# Autodesk Inventor assembly: XL430-bracket
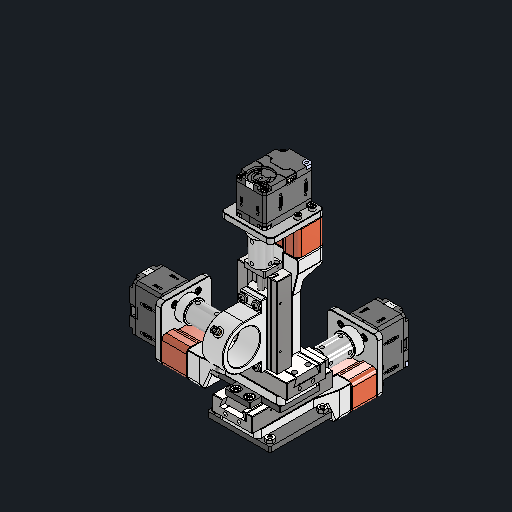
[picture p0: Inventor's stored thumbnail of the model, 512x512]
Saved by Autodesk Inventor 2027.1 (Build 311270010, 270A)
## iProperties
Created: 2025-05-28
Part Number: XL430-bracket
Document SubType Name: Assembly
Designer: kuzmin
Mass: 1365.19 g
Surface Area: 1309.73 cm^2
Volume: 325.346 cm^3
Density: 4.19612 g/cm^3
Author: kuzmin
## Documents named in this file (12)
- C:\Users\queezz\Dropbox\Drawings\pihti-cad\LIBS\XL430-bracket.iam
- C:\Users\queezz\Dropbox\Drawings\pihti-cad\LIBS\TAS-20605L\TAS-60-09B.ipt
- C:\Users\queezz\Dropbox\Drawings\pihti-cad\LIBS\TAS-20605L\TAS-dovegroove.ipt
- C:\Users\queezz\Dropbox\Drawings\pihti-cad\LIBS\TAS-20605L\TAS-60XYZ-Y-slider.ipt
- C:\Users\queezz\Dropbox\Drawings\pihti-cad\LIBS\TAS-20605L\TAS-60XYZ-cross-plate.ipt
- C:\Users\queezz\Dropbox\Drawings\pihti-cad\LIBS\Motor-Bracket-with-inserts.iam
- C:\Users\queezz\Dropbox\Drawings\pihti-cad\ContentCenter\Fastners\M4x10-SHCS.ipt
- C:\Users\queezz\Dropbox\Drawings\pihti-cad\ContentCenter\Fastners\M4x12-Fillips-Countersink.ipt
- C:\Users\queezz\Dropbox\Drawings\pihti-cad\LIBS\TAS-20605L\TAS-60XYZ-mounting-plate.ipt
- C:\Users\queezz\Dropbox\Drawings\pihti-cad\ContentCenter\Fastners\M4-nut.ipt
- C:\Users\queezz\Dropbox\Drawings\pihti-cad\ContentCenter\Fastners\M4x10-fillips-round.ipt
- C:\Users\queezz\Dropbox\Drawings\pihti-cad\LIBS\lens-clamp-hsi.iam
## Components (32 placed, 11 different names)
1. TAS-60-09B:1 — Mate:4, Flush:1, Flush:7, Flush:8
2. TAS-dovegroove:1 — Mate:4, Flush:1, Rigid:3, Flush:7, Flush:8, Rigid:22
3. TAS-60-09B:2 — Flush:3, Mate:9, Flush:5, Rigid:31
4. TAS-dovegroove:2 — Flush:3, Mate:9, Flush:5, Rigid:23
5. TAS-dovegroove:3 — Flush:2, Mate:8, Flush:9, Rigid:25
6. TAS-60XYZ-Y-slider:1 — Flush:2, Mate:8, Rigid:3, Flush:9
7. TAS-60XYZ-cross-plate:1 — Rigid:27, Rigid:28, Rigid:29, Rigid:30, Rigid:26, Rigid:31
8. Motor-Bracket-with-inserts:1 [sub-assembly] — Rigid:22, Rotational:7, Rotational:8, Rotational:9, Rotational:10
9. Motor-Bracket-with-inserts:2 [sub-assembly] — Rigid:25, Rigid:26
10. Motor-Bracket-with-inserts:3 [sub-assembly] — Rigid:21, Rigid:23
11. TAS-60XYZ-mounting-plate:1 — Rigid:13, Rigid:14, Rigid:15, Rigid:16, Rigid:17, Rigid:18, Rigid:19, Rigid:20, Rigid:21
12. lens-clamp-hsi:1 [sub-assembly]
13. BS EN ISO 7045 H - Metric M4 x 10 - 4.8 - H:1
14. BS EN ISO 7045 H - Metric M4 x 10 - 4.8 - H:2
15. BS EN ISO 7045 H - Metric M4 x 10 - 4.8 - H:3
16. BS EN ISO 7045 H - Metric M4 x 10 - 4.8 - H:4
17. JIS B 1181 -finished Class 1 - Metric Class 1 -finishedM4:1 — Rigid:20
18. JIS B 1181 -finished Class 1 - Metric Class 1 -finishedM4:2 — Rigid:19
19. JIS B 1181 -finished Class 1 - Metric Class 1 -finishedM4:3 — Rigid:18
20. JIS B 1181 -finished Class 1 - Metric Class 1 -finishedM4:4 — Rigid:17
21. AS 1427 Z - Metric M4 x 12:5 — Rigid:14
22. AS 1427 Z - Metric M4 x 12:6 — Rigid:16
23. AS 1427 Z - Metric M4 x 12:7 — Rigid:15
24. AS 1427 Z - Metric M4 x 12:8 — Rigid:13
25. AS 1427 Z - Metric M4 x 12:1 — Rigid:29
26. AS 1427 Z - Metric M4 x 12:2 — Rigid:28
27. AS 1427 Z - Metric M4 x 12:3 — Rigid:27
28. AS 1427 Z - Metric M4 x 12:4 — Rigid:30
29. AS 1420 - Metric M4 x 10:1 — Rotational:8
30. AS 1420 - Metric M4 x 10:2 — Rotational:7
31. AS 1420 - Metric M4 x 10:3 — Rotational:9
32. AS 1420 - Metric M4 x 10:4 — Rotational:10
## Relationships (38: WeldJoint 24, Flush 7, RevoluteJoint 4, Mate 3)
- Mate:4: TAS-60-09B:1 ↔ TAS-dovegroove:1
- Flush:1: TAS-60-09B:1 ↔ TAS-dovegroove:1
- Flush:2: TAS-dovegroove:3 ↔ TAS-60XYZ-Y-slider:1
- Mate:8: TAS-dovegroove:3 ↔ TAS-60XYZ-Y-slider:1
- Flush:3: TAS-60-09B:2 ↔ TAS-dovegroove:2
- Mate:9: TAS-60-09B:2 ↔ TAS-dovegroove:2
- Rigid:3 [WeldJoint]: TAS-dovegroove:1 ↔ TAS-60XYZ-Y-slider:1
- Flush:5: TAS-60-09B:2 ↔ TAS-dovegroove:2
- Flush:7: TAS-60-09B:1 ↔ TAS-dovegroove:1
- Flush:8: TAS-60-09B:1 ↔ TAS-dovegroove:1
- Flush:9: TAS-dovegroove:3 ↔ TAS-60XYZ-Y-slider:1
- Rigid:27 [WeldJoint]: TAS-60XYZ-cross-plate:1 ↔ AS 1427 Z - Metric M4 x 12:3
- Rigid:28 [WeldJoint]: TAS-60XYZ-cross-plate:1 ↔ AS 1427 Z - Metric M4 x 12:2
- Rigid:29 [WeldJoint]: TAS-60XYZ-cross-plate:1 ↔ AS 1427 Z - Metric M4 x 12:1
- Rigid:30 [WeldJoint]: TAS-60XYZ-cross-plate:1 ↔ AS 1427 Z - Metric M4 x 12:4
- Rigid:13 [WeldJoint]: TAS-60XYZ-mounting-plate:1 ↔ AS 1427 Z - Metric M4 x 12:8
- Rigid:14 [WeldJoint]: TAS-60XYZ-mounting-plate:1 ↔ AS 1427 Z - Metric M4 x 12:5
- Rigid:15 [WeldJoint]: TAS-60XYZ-mounting-plate:1 ↔ AS 1427 Z - Metric M4 x 12:7
- Rigid:16 [WeldJoint]: TAS-60XYZ-mounting-plate:1 ↔ AS 1427 Z - Metric M4 x 12:6
- Rigid:17 [WeldJoint]: TAS-60XYZ-mounting-plate:1 ↔ JIS B 1181 -finished Class 1 - Metric Class 1 -finishedM4:4
- Rigid:18 [WeldJoint]: TAS-60XYZ-mounting-plate:1 ↔ JIS B 1181 -finished Class 1 - Metric Class 1 -finishedM4:3
- Rigid:19 [WeldJoint]: TAS-60XYZ-mounting-plate:1 ↔ JIS B 1181 -finished Class 1 - Metric Class 1 -finishedM4:2
- Rigid:20 [WeldJoint]: TAS-60XYZ-mounting-plate:1 ↔ JIS B 1181 -finished Class 1 - Metric Class 1 -finishedM4:1
- Rigid:21 [WeldJoint]: Motor-Bracket-with-inserts:3 ↔ TAS-60XYZ-mounting-plate:1
- Rigid:22 [WeldJoint]: TAS-dovegroove:1 ↔ Motor-Bracket-with-inserts:1
- Rigid:23 [WeldJoint]: TAS-dovegroove:2 ↔ Motor-Bracket-with-inserts:3
- Rigid:25 [WeldJoint]: TAS-dovegroove:3 ↔ Motor-Bracket-with-inserts:2
- Rigid:26 [WeldJoint]: TAS-60XYZ-cross-plate:1 ↔ Motor-Bracket-with-inserts:2
- [WeldJoint]: TAS-60-09B:1 ↔ lens-clamp-hsi:1
- Rotational:7 [RevoluteJoint]: Motor-Bracket-with-inserts:1 ↔ AS 1420 - Metric M4 x 10:2
- Rotational:8 [RevoluteJoint]: Motor-Bracket-with-inserts:1 ↔ AS 1420 - Metric M4 x 10:1
- Rotational:9 [RevoluteJoint]: Motor-Bracket-with-inserts:1 ↔ AS 1420 - Metric M4 x 10:3
- Rotational:10 [RevoluteJoint]: Motor-Bracket-with-inserts:1 ↔ AS 1420 - Metric M4 x 10:4
- Rigid:31 [WeldJoint]: TAS-60-09B:2 ↔ TAS-60XYZ-cross-plate:1
- [WeldJoint]: lens-clamp-hsi:1 ↔ BS EN ISO 7045 H - Metric M4 x 10 - 4.8 - H:4
- [WeldJoint]: lens-clamp-hsi:1 ↔ BS EN ISO 7045 H - Metric M4 x 10 - 4.8 - H:2
- [WeldJoint]: lens-clamp-hsi:1 ↔ BS EN ISO 7045 H - Metric M4 x 10 - 4.8 - H:1
- [WeldJoint]: lens-clamp-hsi:1 ↔ BS EN ISO 7045 H - Metric M4 x 10 - 4.8 - H:3
